# Autodesk Inventor assembly: JukeBoxAssembly_Ocampo_COLORED
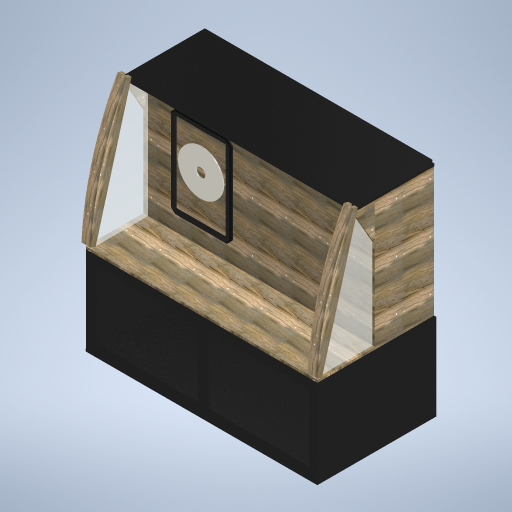
[picture p0: Inventor's stored thumbnail of the model, 512x512]
Saved by Autodesk Inventor 2023 (Build 270158000, 158)
## iProperties
Created: 2025-03-05
Part Number: JukeBoxAssembly_Ocampo_COLORED
Document SubType Name: Assembly
Designer: FrameUser
Author: FrameUser
## Documents named in this file (13)
- G:\My Drive\Digital Electronics\JukeBoxAssembly_Ocampo_COLORED.iam
- G:\My Drive\Digital Electronics\BottomOfTheBottomOfTheJukebox_Ocampo.ipt
- G:\My Drive\Digital Electronics\BottomHalfofSides_Ocampo.ipt
- G:\My Drive\Digital Electronics\BottomHalfofFront_Ocampo.ipt
- G:\My Drive\Digital Electronics\UpperHalfofSides_Ocampo.ipt
- G:\My Drive\Digital Electronics\Triangle_Ocampo.ipt
- G:\My Drive\Digital Electronics\TopOfTheBottomOftheJukebox_Ocampo.ipt
- G:\My Drive\Digital Electronics\TopOfTheTopOfTheJukebox_Ocampo.ipt
- G:\My Drive\Digital Electronics\UpperHalfofFrontBack_Ocampo.ipt
- G:\My Drive\Digital Electronics\BottomHalfOfBack.ipt
- G:\My Drive\Digital Electronics\glass_Ocampo.ipt
- G:\My Drive\Digital Electronics\CD_Ocampo.ipt
- G:\My Drive\Digital Electronics\sidestrip_Ocampo.ipt
## Components (18 placed, 12 different names)
1. BottomOfTheBottomOfTheJukebox_Ocampo:1 — Mate:1, Flush:1, Flush:2, Mate:2, Flush:3, Flush:4, Mate:3, Flush:5, Flush:23
2. BottomHalfofSides_Ocampo:1 — Mate:1, Flush:1, Flush:2, Mate:5, Flush:6, Flush:7, Mate:13
3. BottomHalfofSides_Ocampo:2 — Mate:2, Flush:3, Flush:4, Mate:4, Mate:6, Flush:8, Flush:9, Mate:9, Flush:15, Flush:22
4. BottomHalfofFront_Ocampo:1 — Mate:3, Flush:5, Mate:4, Flush:14
5. UpperHalfofSides_Ocampo:1 — Mate:5, Flush:6, Flush:7, Mate:8, Flush:12, Flush:13, Flush:18, Flush:19, Mate:12, Mate:17
6. UpperHalfofSides_Ocampo:2 — Mate:6, Flush:8, Flush:9, Mate:7, Flush:10, Flush:11, Mate:10, Flush:16, Flush:17, Mate:11, Flush:20
7. Triangle_Ocampo:1 — Mate:7, Flush:10, Flush:11, Mate:15
8. Triangle_Ocampo:2 — Mate:8, Flush:12, Flush:13, Flush:24
9. TopOfTheBottomOftheJukebox_Ocampo:1 — Mate:9, Flush:14, Flush:15
10. TopOfTheTopOfTheJukebox_Ocampo:1 — Mate:10, Flush:16, Flush:17, Flush:21, Mate:16, Flush:25
11. UpperHalfofFrontBack_Ocampo:1 — Mate:11, Flush:18, Flush:19, Mate:14, Mate:18, Mate:19
12. UpperHalfofFrontBack_Ocampo:2 — Mate:12, Flush:20, Flush:21
13. BottomHalfOfBack:1 — Mate:13, Flush:22, Flush:23
14. glass_Ocampo:1 — Mate:14, Mate:15, Mate:16, Mate:20, Mate:21
15. glass_Ocampo:2 — Flush:24, Mate:17, Flush:25, Mate:22, Mate:23
16. CD_Ocampo:1 — Mate:18, Mate:19
17. sidestrip_Ocampo:1 — Mate:20, Mate:21
18. sidestrip_Ocampo:2 — Mate:22, Mate:23
## Relationships (48: Flush 25, Mate 23)
- Mate:1: BottomOfTheBottomOfTheJukebox_Ocampo:1 ↔ BottomHalfofSides_Ocampo:1
- Flush:1: BottomOfTheBottomOfTheJukebox_Ocampo:1 ↔ BottomHalfofSides_Ocampo:1
- Flush:2: BottomOfTheBottomOfTheJukebox_Ocampo:1 ↔ BottomHalfofSides_Ocampo:1
- Mate:2: BottomOfTheBottomOfTheJukebox_Ocampo:1 ↔ BottomHalfofSides_Ocampo:2
- Flush:3: BottomOfTheBottomOfTheJukebox_Ocampo:1 ↔ BottomHalfofSides_Ocampo:2
- Flush:4: BottomOfTheBottomOfTheJukebox_Ocampo:1 ↔ BottomHalfofSides_Ocampo:2
- Mate:3: BottomOfTheBottomOfTheJukebox_Ocampo:1 ↔ BottomHalfofFront_Ocampo:1
- Flush:5: BottomOfTheBottomOfTheJukebox_Ocampo:1 ↔ BottomHalfofFront_Ocampo:1
- Mate:4: BottomHalfofSides_Ocampo:2 ↔ BottomHalfofFront_Ocampo:1
- Mate:5: BottomHalfofSides_Ocampo:1 ↔ UpperHalfofSides_Ocampo:1
- Flush:6: BottomHalfofSides_Ocampo:1 ↔ UpperHalfofSides_Ocampo:1
- Flush:7: BottomHalfofSides_Ocampo:1 ↔ UpperHalfofSides_Ocampo:1
- Mate:6: BottomHalfofSides_Ocampo:2 ↔ UpperHalfofSides_Ocampo:2
- Flush:8: BottomHalfofSides_Ocampo:2 ↔ UpperHalfofSides_Ocampo:2
- Flush:9: BottomHalfofSides_Ocampo:2 ↔ UpperHalfofSides_Ocampo:2
- Mate:7: UpperHalfofSides_Ocampo:2 ↔ Triangle_Ocampo:1
- Flush:10: UpperHalfofSides_Ocampo:2 ↔ Triangle_Ocampo:1
- Flush:11: UpperHalfofSides_Ocampo:2 ↔ Triangle_Ocampo:1
- Mate:8: UpperHalfofSides_Ocampo:1 ↔ Triangle_Ocampo:2
- Flush:12: UpperHalfofSides_Ocampo:1 ↔ Triangle_Ocampo:2
- Flush:13: UpperHalfofSides_Ocampo:1 ↔ Triangle_Ocampo:2
- Mate:9: BottomHalfofSides_Ocampo:2 ↔ TopOfTheBottomOftheJukebox_Ocampo:1
- Flush:14: BottomHalfofFront_Ocampo:1 ↔ TopOfTheBottomOftheJukebox_Ocampo:1
- Flush:15: BottomHalfofSides_Ocampo:2 ↔ TopOfTheBottomOftheJukebox_Ocampo:1
- Mate:10: UpperHalfofSides_Ocampo:2 ↔ TopOfTheTopOfTheJukebox_Ocampo:1
- Flush:16: UpperHalfofSides_Ocampo:2 ↔ TopOfTheTopOfTheJukebox_Ocampo:1
- Flush:17: UpperHalfofSides_Ocampo:2 ↔ TopOfTheTopOfTheJukebox_Ocampo:1
- Mate:11: UpperHalfofSides_Ocampo:2 ↔ UpperHalfofFrontBack_Ocampo:1
- Flush:18: UpperHalfofSides_Ocampo:1 ↔ UpperHalfofFrontBack_Ocampo:1
- Flush:19: UpperHalfofSides_Ocampo:1 ↔ UpperHalfofFrontBack_Ocampo:1
- Mate:12: UpperHalfofSides_Ocampo:1 ↔ UpperHalfofFrontBack_Ocampo:2
- Flush:20: UpperHalfofSides_Ocampo:2 ↔ UpperHalfofFrontBack_Ocampo:2
- Flush:21: TopOfTheTopOfTheJukebox_Ocampo:1 ↔ UpperHalfofFrontBack_Ocampo:2
- Mate:13: BottomHalfofSides_Ocampo:1 ↔ BottomHalfOfBack:1
- Flush:22: BottomHalfofSides_Ocampo:2 ↔ BottomHalfOfBack:1
- Flush:23: BottomOfTheBottomOfTheJukebox_Ocampo:1 ↔ BottomHalfOfBack:1
- Mate:14: UpperHalfofFrontBack_Ocampo:1 ↔ glass_Ocampo:1
- Mate:15: Triangle_Ocampo:1 ↔ glass_Ocampo:1
- Mate:16: TopOfTheTopOfTheJukebox_Ocampo:1 ↔ glass_Ocampo:1
- Flush:24 (6.35 mm): Triangle_Ocampo:2 ↔ glass_Ocampo:2
- Mate:17: UpperHalfofSides_Ocampo:1 ↔ glass_Ocampo:2
- Flush:25 (6.35 mm): TopOfTheTopOfTheJukebox_Ocampo:1 ↔ glass_Ocampo:2
- Mate:18: UpperHalfofFrontBack_Ocampo:1 ↔ CD_Ocampo:1
- Mate:19 (69.85 mm): UpperHalfofFrontBack_Ocampo:1 ↔ CD_Ocampo:1
- Mate:20: glass_Ocampo:1 ↔ sidestrip_Ocampo:1
- Mate:21: glass_Ocampo:1 ↔ sidestrip_Ocampo:1
- Mate:22: glass_Ocampo:2 ↔ sidestrip_Ocampo:2
- Mate:23: glass_Ocampo:2 ↔ sidestrip_Ocampo:2
